# Autodesk Inventor assembly: Turret Shooter Assembly
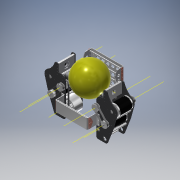
[picture p0: Inventor's stored thumbnail of the model, 180x180]
Saved by Autodesk Inventor 2019.4 (Build 234330000, 330)
## iProperties
Created: 2020-01-06
Part Number: Turret Shooter Assembly
Document SubType Name: Assembly
Designer: admin
Mass: 7599.75 g
Surface Area: 10392.7 cm^2
Volume: 5758.88 cm^3
Density: 1.31966 g/cm^3
Author: admin
## Documents named in this file (26)
- C:\Users\admin\Desktop\FRC 2020 Engineering\GitHub\7738-2020\Turret\Turret Shooter Assembly.iam
- C:\Users\admin\Desktop\FRC 2020 Engineering\GitHub\7738-2020\Turret\Omni Wheel\3_25_Omni-Directional_Wheel_217-4775.iam
- C:\Users\admin\Desktop\FRC 2020 Engineering\GitHub\7738-2020\Power Cell.ipt
- C:\Users\admin\Desktop\FRC 2020 Engineering\GitHub\7738-2020\Turret\Flywheel.ipt
- C:\Users\admin\Desktop\FRC 2020 Engineering\GitHub\7738-2020\Turret\Mini CIM\Mini_CIM_Motor_217-3371.ipt
- C:\Users\admin\Desktop\FRC 2020 Engineering\GitHub\7738-2020\CAD\Gearbox\F6800.ipt
- C:\Users\admin\Desktop\FRC 2020 Engineering\GitHub\7738-2020\Turret\Flywheel Bracket 1.ipt
- C:\Users\admin\Desktop\FRC 2020 Engineering\GitHub\7738-2020\Turret\Pivot Plate.ipt
- C:\Users\admin\Desktop\FRC 2020 Engineering\GitHub\7738-2020\CAD\Gearbox\F6804.ipt
- C:\Users\admin\Desktop\FRC 2020 Engineering\GitHub\7738-2020\Turret\Turret Shooter Assembly\Design Accelerator\Synchronous Belts Transmission6.iam
- C:\Users\admin\Desktop\FRC 2020 Engineering\GitHub\7738-2020\Turret\Turret Shooter Assembly\Design Accelerator\Synchronous Belts Transmission7.iam
- C:\Users\admin\Desktop\FRC 2020 Engineering\GitHub\7738-2020\Turret\Turret Shooter Assembly\Design Accelerator\Synchronous Belts Transmission8.iam
- C:\Users\Mark\Desktop\7738 Helion Engineering\7738-CAD-prep\Butterfly drive\EB38S6 Encoder.ipt
- C:\Users\admin\Desktop\FRC 2020 Engineering\GitHub\7738-2020\Turret\Pivot Plate Idle.ipt
- C:\Users\admin\Desktop\FRC 2020 Engineering\GitHub\7738-2020\Turret\Turret Shooter Assembly\Design Accelerator\Synchronous Belts Transmission9.iam
- C:\Users\admin\Desktop\FRC 2020 Engineering\GitHub\7738-2020\Turret\Turret Shooter Assembly\Design Accelerator\Synchronous Belts Transmission10.iam
- C:\Users\admin\Desktop\FRC 2020 Engineering\GitHub\7738-2020\Turret\Turret Shooter Assembly\Design Accelerator\Synchronous Belts Transmission11.iam
- C:\Users\admin\Desktop\FRC 2020 Engineering\GitHub\7738-2020\Turret\Spacer.ipt
- C:\Users\admin\Desktop\FRC 2020 Engineering\GitHub\7738-2020\Turret\Shooter Spacer.ipt
- C:\Users\admin\Desktop\FRC 2020 Engineering\GitHub\7738-2020\Turret\Roller Bearing.ipt
- C:\Users\admin\Desktop\FRC 2020 Engineering\GitHub\7738-2020\Turret\Bearing Holder.ipt
- C:\Users\admin\Desktop\FRC 2020 Engineering\GitHub\7738-2020\Turret\Roller.ipt
- C:\Users\admin\Desktop\FRC 2020 Engineering\GitHub\7738-2020\Turret\Shooter Spacer Bottom.ipt
- C:\Users\admin\Desktop\FRC 2020 Engineering\GitHub\7738-2020\Turret\Bottom Roler Bearing Holder.ipt
- C:\Users\admin\Desktop\FRC 2020 Engineering\GitHub\7738-2020\Turret\Flywheel Axle.ipt
- C:\Users\admin\Desktop\FRC 2020 Engineering\GitHub\7738-2020\Turret\Omni Axle.ipt
## Components (75 placed, 20 different names)
1. 3_25_Omni-Directional_Wheel_217-4775:1 [sub-assembly] — Mate:5, Mate:6, Flush:3
2. Power Cell:1 — Mate:14, Mate:15, Mate:16
3. Flywheel:1 — Mate:17, Mate:19, Mate:71, Mate:186
4. F6800:2 — Mate:4, Mate:9
5. Flywheel Bracket 1:1 — Mate:3, Mate:4, Mate:7, Mate:8, Mate:9, Mate:13, Angle:1, Mate:28, Flush:1
6. F6800:3 — Mate:27, Mate:183, Mate:184, Mate:185
7. F6800:5 — Mate:6, Mate:7, Mate:8
8. Pivot Plate:1 — Mate:31, Mate:32, Mate:33, Mate:68
9. Mini_CIM_Motor_217-3371:4 — Mate:3, Mate:13, Mate:22, Mate:26
10. Mini_CIM_Motor_217-3371:5 — Mate:22, Mate:23, Mate:24, Mate:25
11. Flywheel Bracket 1:2 — Mate:24, Mate:25, Mate:26, Mate:27, Mate:28, Mate:29, Mate:30, Mate:31, Mate:32, Mate:33, Flush:2, Mate:73, Mate:74, Mate:76, Mate:77, Mate:78, Mate:79, Mate:80, Mate:81, Flush:5, Flush:6, Mate:133, Mate:134, Mate:185
12. F6800:6 — Mate:29, Mate:30, Mate:187, Mate:188
13. Synchronous Belts Transmission:1 [sub-assembly]
14. Synchronous Belts Transmission:2 [sub-assembly]
15. Synchronous Belts Transmission:3 [sub-assembly]
16. EB38S6 Encoder:1 — Mate:133, Mate:134
17. Flywheel Bracket 1:3 — Mate:49, Mate:52, Mate:53, Mate:56, Mate:57, Mate:58, Mate:61, Mate:62, Mate:65, Mate:66, Mate:137, Flush:7, Flush:8
18. Flywheel Bracket 1:4 — Mate:50, Mate:51, Mate:53, Mate:54, Mate:55, Mate:57, Mate:58, Mate:59, Mate:60, Mate:63, Mate:64, Flush:2, Mate:83, Mate:84, Mate:85, Mate:86, Mate:87, Mate:88, Mate:89, Mate:90, Mate:91, Mate:92, Mate:93, Mate:135, Mate:136
19. Flywheel:2 — Mate:71, Mate:72
20. 3_25_Omni-Directional_Wheel_217-4775:2 [sub-assembly] — Mate:67, Flush:4
21. Pivot Plate Idle:1 — Mate:54, Mate:55, Mate:56, Mate:68, Mate:179, Mate:180
22. Mini_CIM_Motor_217-3371:8 — Mate:49, Mate:52
23. Mini_CIM_Motor_217-3371:9 — Mate:50, Mate:51
24. F6800:7 — Mate:60, Mate:63, Mate:67, Mate:191, Mate:192
25. F6800:8 — Mate:62, Mate:66
26. F6800:9 — Mate:59, Mate:64, Mate:189, Mate:190
27. F6800:10 — Mate:61, Mate:65
28. Synchronous Belts Transmission:4 [sub-assembly]
29. Synchronous Belts Transmission:5 [sub-assembly]
30. Synchronous Belts Transmission:6 [sub-assembly]
31. Spacer:1 — Mate:73, Mate:80
32. Spacer:3 — Mate:74, Mate:81
33. Spacer:5 — Mate:76, Mate:79
34. Spacer:6 — Mate:77, Mate:78
35. Spacer:7 — Mate:83, Mate:89
36. Spacer:8 — Mate:84, Mate:90
37. Spacer:9 — Mate:85, Mate:91
38. Spacer:10 — Mate:86, Mate:92
39. Spacer:11 — Mate:87, Mate:88
40. Shooter Spacer:1 — Mate:93, Flush:5, Flush:6, Mate:94, Mate:95, Mate:96, Mate:171, Mate:177, Mate:178
41. Roller Bearing:3 — Mate:100, Mate:109, Mate:127
42. Bearing Holder:1 — Mate:94, Mate:95, Mate:96, Mate:100, Mate:101, Mate:103, Mate:104, Mate:105, Mate:106, Mate:107, Mate:108, Mate:109, Mate:156, Mate:157, Mate:158
43. Roller Bearing:5 — Mate:107, Mate:125, Mate:156
44. Roller Bearing:6 — Mate:103, Mate:106, Mate:124
45. Roller Bearing:7 — Mate:104, Mate:105, Mate:123
46. Roller Bearing:8 — Mate:101, Mate:108, Mate:126
47. Roller:1 — Mate:127, Mate:176
48. Roller:2 — Mate:126, Mate:175
49. Roller:3 — Mate:125, Mate:174
50. Roller:4 — Mate:124, Mate:173
51. Roller:5 — Mate:123, Mate:172
52. EB38S6 Encoder:2 — Mate:135, Mate:136
53. Shooter Spacer Bottom:1 — Mate:137, Flush:7, Flush:8, Mate:142, Mate:143, Mate:144, Mate:149, Mate:150, Mate:151
54. Bottom Roler Bearing Holder:1 — Mate:138, Mate:139, Mate:140, Mate:141, Mate:142, Mate:143, Mate:144
55. Roller Bearing:14 — Mate:138, Mate:140, Mate:154
56. Roller Bearing:15 — Mate:139, Mate:141, Mate:155
57. Bottom Roler Bearing Holder:2 — Mate:149, Mate:150, Mate:151
58. Roller Bearing:16 — Mate:152
59. Roller Bearing:17 — Mate:153
60. Roller:6 — Mate:152, Mate:155
61. Roller:7 — Mate:153, Mate:154
62. Roller Bearing:18 — Mate:157, Mate:158, Mate:181
63. Roller Bearing:19 — Mate:172
64. Bearing Holder:2 — Mate:171, Mate:177, Mate:178
65. Roller Bearing:20 — Mate:182
66. Roller Bearing:21 — Mate:175
67. Roller Bearing:22 — Mate:176
68. Roller Bearing:23 — Mate:173
69. Roller Bearing:24 — Mate:174
70. F6804:1 — Mate:179, Mate:180
71. Roller:8 — Mate:181, Mate:182
72. Flywheel Axle:1 — Mate:183, Mate:184, Mate:186
73. Omni Axle:1 — Mate:187, Mate:188
74. Flywheel Axle:2 — Mate:189, Mate:190
75. Omni Axle:2 — Mate:191, Mate:192
## Relationships (154: Mate 145, Flush 8, Angle 1)
- Mate:3: Flywheel Bracket 1:1 ↔ Mini_CIM_Motor_217-3371:4
- Mate:4: F6800:2 ↔ Flywheel Bracket 1:1
- Mate:5: 3_25_Omni-Directional_Wheel_217-4775:1
- Mate:6: 3_25_Omni-Directional_Wheel_217-4775:1 ↔ F6800:5
- Mate:7: Flywheel Bracket 1:1 ↔ F6800:5
- Mate:8 (0.2 mm): Flywheel Bracket 1:1 ↔ F6800:5
- Mate:9 (0.2 mm): F6800:2 ↔ Flywheel Bracket 1:1
- Mate:13: Flywheel Bracket 1:1 ↔ Mini_CIM_Motor_217-3371:4
- Mate:14: Power Cell:1
- Mate:15: Power Cell:1
- Mate:16: Power Cell:1
- Mate:17 (104.775 mm): Flywheel:1
- Mate:18 (104.775 mm)
- Angle:1 (0 deg): Flywheel Bracket 1:1
- Mate:19 (-25 mm): Flywheel:1
- Mate:20 (-65 mm)
- Mate:22 (72.5 mm): Mini_CIM_Motor_217-3371:4 ↔ Mini_CIM_Motor_217-3371:5
- Mate:23 (77.5 mm): Mini_CIM_Motor_217-3371:5
- Mate:24: Mini_CIM_Motor_217-3371:5 ↔ Flywheel Bracket 1:2
- Mate:25: Mini_CIM_Motor_217-3371:5 ↔ Flywheel Bracket 1:2
- Mate:26: Mini_CIM_Motor_217-3371:4 ↔ Flywheel Bracket 1:2
- Mate:27 (0.2 mm): F6800:3 ↔ Flywheel Bracket 1:2
- Mate:28 (95 mm): Flywheel Bracket 1:1 ↔ Flywheel Bracket 1:2
- Flush:1 (47.5 mm): Flywheel Bracket 1:1
- Mate:29: Flywheel Bracket 1:2 ↔ F6800:6
- Mate:30 (0.2 mm): Flywheel Bracket 1:2 ↔ F6800:6
- Mate:31: Pivot Plate:1 ↔ Flywheel Bracket 1:2
- Mate:32: Pivot Plate:1 ↔ Flywheel Bracket 1:2
- Mate:33: Pivot Plate:1 ↔ Flywheel Bracket 1:2
- Mate:49: Flywheel Bracket 1:3 ↔ Mini_CIM_Motor_217-3371:8
- Mate:50: Flywheel Bracket 1:4 ↔ Mini_CIM_Motor_217-3371:9
- Mate:51: Flywheel Bracket 1:4 ↔ Mini_CIM_Motor_217-3371:9
- Mate:52: Flywheel Bracket 1:3 ↔ Mini_CIM_Motor_217-3371:8
- Mate:53 (95 mm): Flywheel Bracket 1:3 ↔ Flywheel Bracket 1:4
- Mate:54: Flywheel Bracket 1:4 ↔ Pivot Plate Idle:1
- Mate:55: Flywheel Bracket 1:4 ↔ Pivot Plate Idle:1
- Mate:56: Flywheel Bracket 1:3 ↔ Pivot Plate Idle:1
- Mate:57: Flywheel Bracket 1:3 ↔ Flywheel Bracket 1:4
- Mate:58: Flywheel Bracket 1:3 ↔ Flywheel Bracket 1:4
- Mate:59: Flywheel Bracket 1:4 ↔ F6800:9
- Mate:60: Flywheel Bracket 1:4 ↔ F6800:7
- Mate:61: Flywheel Bracket 1:3 ↔ F6800:10
- Mate:62: Flywheel Bracket 1:3 ↔ F6800:8
- Mate:63 (0.2 mm): Flywheel Bracket 1:4 ↔ F6800:7
- Mate:64 (0.2 mm): Flywheel Bracket 1:4 ↔ F6800:9
- Mate:65 (0.2 mm): Flywheel Bracket 1:3 ↔ F6800:10
- Mate:66 (0.2 mm): Flywheel Bracket 1:3 ↔ F6800:8
- Mate:67: 3_25_Omni-Directional_Wheel_217-4775:2 ↔ F6800:7
- Mate:68: Pivot Plate:1 ↔ Pivot Plate Idle:1
- Flush:2: Flywheel Bracket 1:2 ↔ Flywheel Bracket 1:4
- Mate:71 (209.55 mm): Flywheel:1 ↔ Flywheel:2
- Mate:72 (-25 mm): Flywheel:2
- Flush:3 (-19.05 mm): 3_25_Omni-Directional_Wheel_217-4775:1
- Flush:4 (-19.05 mm): 3_25_Omni-Directional_Wheel_217-4775:2
- Mate:73: Flywheel Bracket 1:2 ↔ Spacer:1
- Mate:74: Flywheel Bracket 1:2 ↔ Spacer:3
- Mate:76: Flywheel Bracket 1:2 ↔ Spacer:5
- Mate:77: Flywheel Bracket 1:2 ↔ Spacer:6
- Mate:78: Flywheel Bracket 1:2 ↔ Spacer:6
- Mate:79: Flywheel Bracket 1:2 ↔ Spacer:5
- Mate:80: Flywheel Bracket 1:2 ↔ Spacer:1
- Mate:81: Flywheel Bracket 1:2 ↔ Spacer:3
- Mate:83: Flywheel Bracket 1:4 ↔ Spacer:7
- Mate:84: Flywheel Bracket 1:4 ↔ Spacer:8
- Mate:85: Flywheel Bracket 1:4 ↔ Spacer:9
- Mate:86: Flywheel Bracket 1:4 ↔ Spacer:10
- Mate:87: Flywheel Bracket 1:4 ↔ Spacer:11
- Mate:88: Flywheel Bracket 1:4 ↔ Spacer:11
- Mate:89: Flywheel Bracket 1:4 ↔ Spacer:7
- Mate:90: Flywheel Bracket 1:4 ↔ Spacer:8
- Mate:91: Flywheel Bracket 1:4 ↔ Spacer:9
- Mate:92: Flywheel Bracket 1:4 ↔ Spacer:10
- Mate:93: Flywheel Bracket 1:4 ↔ Shooter Spacer:1
- Flush:5 (70 mm): Flywheel Bracket 1:2 ↔ Shooter Spacer:1
- Flush:6: Flywheel Bracket 1:2 ↔ Shooter Spacer:1
- Mate:94: Shooter Spacer:1 ↔ Bearing Holder:1
- Mate:95: Shooter Spacer:1 ↔ Bearing Holder:1
- Mate:96 (0.2 mm): Shooter Spacer:1 ↔ Bearing Holder:1
- Mate:100: Roller Bearing:3 ↔ Bearing Holder:1
- Mate:101: Bearing Holder:1 ↔ Roller Bearing:8
- Mate:103: Bearing Holder:1 ↔ Roller Bearing:6
- Mate:104: Bearing Holder:1 ↔ Roller Bearing:7
- Mate:105 (0.2 mm): Bearing Holder:1 ↔ Roller Bearing:7
- Mate:106 (0.2 mm): Bearing Holder:1 ↔ Roller Bearing:6
- Mate:107 (0.2 mm): Bearing Holder:1 ↔ Roller Bearing:5
- Mate:108 (0.2 mm): Bearing Holder:1 ↔ Roller Bearing:8
- Mate:109 (0.2 mm): Roller Bearing:3 ↔ Bearing Holder:1
- Mate:123: Roller Bearing:7 ↔ Roller:5
- Mate:124: Roller Bearing:6 ↔ Roller:4
- Mate:125: Roller Bearing:5 ↔ Roller:3
- Mate:126: Roller Bearing:8 ↔ Roller:2
- Mate:127: Roller Bearing:3 ↔ Roller:1
- Mate:133: Flywheel Bracket 1:2 ↔ EB38S6 Encoder:1
- Mate:134: Flywheel Bracket 1:2 ↔ EB38S6 Encoder:1
- Mate:135: Flywheel Bracket 1:4 ↔ EB38S6 Encoder:2
- Mate:136: Flywheel Bracket 1:4 ↔ EB38S6 Encoder:2
- Mate:137: Flywheel Bracket 1:3 ↔ Shooter Spacer Bottom:1
- Flush:7 (70 mm): Flywheel Bracket 1:3 ↔ Shooter Spacer Bottom:1
- Flush:8: Flywheel Bracket 1:3 ↔ Shooter Spacer Bottom:1
- Mate:138: Bottom Roler Bearing Holder:1 ↔ Roller Bearing:14
- Mate:139: Bottom Roler Bearing Holder:1 ↔ Roller Bearing:15
- Mate:140 (0.2 mm): Bottom Roler Bearing Holder:1 ↔ Roller Bearing:14
- Mate:141 (0.2 mm): Bottom Roler Bearing Holder:1 ↔ Roller Bearing:15
- Mate:142 (0.2 mm): Shooter Spacer Bottom:1 ↔ Bottom Roler Bearing Holder:1
- Mate:143: Shooter Spacer Bottom:1 ↔ Bottom Roler Bearing Holder:1
- Mate:144: Shooter Spacer Bottom:1 ↔ Bottom Roler Bearing Holder:1
- [Mate]: Bottom Roler Bearing Holder:2 ↔ Roller Bearing:16
- [Mate]: Bottom Roler Bearing Holder:2 ↔ Roller Bearing:17
- [Mate] (0.2 mm): Bottom Roler Bearing Holder:2 ↔ Roller Bearing:16
- [Mate] (0.2 mm): Bottom Roler Bearing Holder:2 ↔ Roller Bearing:17
- Mate:149 (0.2 mm): Shooter Spacer Bottom:1 ↔ Bottom Roler Bearing Holder:2
- Mate:150: Shooter Spacer Bottom:1 ↔ Bottom Roler Bearing Holder:2
- Mate:151: Shooter Spacer Bottom:1 ↔ Bottom Roler Bearing Holder:2
- Mate:152: Roller Bearing:16 ↔ Roller:6
- Mate:153: Roller Bearing:17 ↔ Roller:7
- Mate:154 (0.2 mm): Roller Bearing:14 ↔ Roller:7
- Mate:155 (0.2 mm): Roller Bearing:15 ↔ Roller:6
- Mate:156: Bearing Holder:1 ↔ Roller Bearing:5
- Mate:157: Bearing Holder:1 ↔ Roller Bearing:18
- Mate:158 (0.2 mm): Bearing Holder:1 ↔ Roller Bearing:18
- [Mate]: Roller Bearing:19 ↔ Bearing Holder:2
- [Mate]: Bearing Holder:2 ↔ Roller Bearing:23
- [Mate]: Bearing Holder:2 ↔ Roller Bearing:21
- [Mate]: Bearing Holder:2 ↔ Roller Bearing:22
- [Mate] (0.2 mm): Bearing Holder:2 ↔ Roller Bearing:22
- [Mate] (0.2 mm): Bearing Holder:2 ↔ Roller Bearing:21
- [Mate] (0.2 mm): Bearing Holder:2 ↔ Roller Bearing:20
- [Mate] (0.2 mm): Bearing Holder:2 ↔ Roller Bearing:23
- [Mate] (0.2 mm): Roller Bearing:19 ↔ Bearing Holder:2
- [Mate]: Bearing Holder:2 ↔ Roller Bearing:20
- [Mate]: Bearing Holder:2 ↔ Roller Bearing:24
- [Mate] (0.2 mm): Bearing Holder:2 ↔ Roller Bearing:24
- Mate:171 (0.2 mm): Shooter Spacer:1 ↔ Bearing Holder:2
- Mate:172 (0.2 mm): Roller:5 ↔ Roller Bearing:19
- Mate:173 (0.2 mm): Roller:4 ↔ Roller Bearing:23
- Mate:174 (0.2 mm): Roller:3 ↔ Roller Bearing:24
- Mate:175 (0.2 mm): Roller:2 ↔ Roller Bearing:21
- Mate:176 (0.2 mm): Roller:1 ↔ Roller Bearing:22
- Mate:177: Shooter Spacer:1 ↔ Bearing Holder:2
- Mate:178: Shooter Spacer:1 ↔ Bearing Holder:2
- Mate:179: Pivot Plate Idle:1 ↔ F6804:1
- Mate:180 (0.2 mm): Pivot Plate Idle:1 ↔ F6804:1
- Mate:181: Roller Bearing:18 ↔ Roller:8
- Mate:182 (0.2 mm): Roller Bearing:20 ↔ Roller:8
- Mate:183: F6800:3 ↔ Flywheel Axle:1
- Mate:184 (0.1 mm): F6800:3 ↔ Flywheel Axle:1
- Mate:185: F6800:3 ↔ Flywheel Bracket 1:2
- Mate:186: Flywheel:1 ↔ Flywheel Axle:1
- Mate:187: F6800:6 ↔ Omni Axle:1
- Mate:188 (0.1 mm): F6800:6 ↔ Omni Axle:1
- Mate:189 (0.1 mm): F6800:9 ↔ Flywheel Axle:2
- Mate:190: F6800:9 ↔ Flywheel Axle:2
- Mate:191: F6800:7 ↔ Omni Axle:2
- Mate:192 (0.1 mm): F6800:7 ↔ Omni Axle:2
## Named parameters: d342_d338 = 0.2 mm, d343_d336 = 0 mm, d344_d337 = 0.2 mm, d345_d335 = 0 mm, d356_d355 = 0.2 mm, d357_d354 = 0 mm, d358_d353 = 0 mm, d359_d299 = 0 mm, d360_d298 = 0 mm, d361_d296 = 0 mm, d362_d304 = 0.2 mm, d363_d303 = 0.2 mm, d364_d302 = 0.2 mm, d365_d301 = 0.2 mm, d366_d300 = 0.2 mm, d367_d294 = 0 mm
